# Autodesk Inventor assembly: switchplate-2
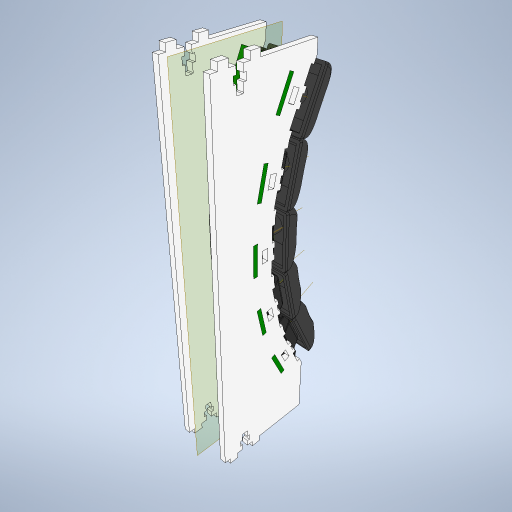
[picture p0: Inventor's stored thumbnail of the model, 512x512]
Saved by Autodesk Inventor 2024.1 (Build 281209000, 209)
## iProperties
Created: 2019-07-06
Part Number: switchplate-2
Document SubType Name: Assembly
Designer: Thibault
Mass: 36.7321 g
Surface Area: 336.688 cm^2
Volume: 13.7102 cm^3
Density: 2.67918 g/cm^3
Author: Thibault
## Documents named in this file (7)
- C:\Users\Thibault\Documents\habilis\mech\switchplate\switchplate-2.iam
- C:\Users\Thibault\Documents\habilis\mech\switchplate_support.ipt
- C:\Users\Thibault Polge\Documents\Habilis\mech\mx.iam
- C:\Users\Thibault\Documents\habilis\mech\mx\DSA-1x1.iam
- C:\Users\Thibault\Documents\habilis\mech\pcb.ipt
- C:\Users\Thibault\Documents\habilis\mech\switchplate.iam
- C:\Users\Thibault\Documents\habilis\mech\switchplate_support\switchplate-support-02.ipt
## Components (12 placed, 4 different names)
1. switchplate-support:left — Affleurement:1, Affleurement:2, Affleurement:3, Affleurement:17, Symétrie:1, Affleurement:23, Placage:1, Placage:3, Placage:6, Placage:7
2. switchplate-support:right — Affleurement:17, Symétrie:1, Affleurement:23, Placage:2, Placage:4, Placage:5, Placage:6, Placage:8, Placage:9, Placage:10, Placage:12, Placage:13, Placage:14, Placage:15, Placage:16, Placage:17, Placage:18, Placage:19, Placage:20, Placage:21, Placage:22, Placage:23, Placage:24, Placage:25, Placage:26, Placage:27, Placage:28, Placage:29, Placage:30, Placage:31, Placage:32
3. Switch:1 [sub-assembly] — Placage:1, Placage:2, Placage:3
4. Switch:2 [sub-assembly] — Placage:8, Placage:9, Placage:10
5. Switch:3 [sub-assembly] — Placage:4, Placage:5, Placage:7
6. Switch:4 [sub-assembly] — Placage:12, Placage:13, Placage:14
7. Switch:5 [sub-assembly] — Placage:15, Placage:16, Placage:17
8. pcb:1 — Placage:21, Placage:31, Placage:32
9. pcb:2 — Placage:22, Placage:29, Placage:30
10. pcb:3 — Placage:19, Placage:27, Placage:28
11. pcb:5 — Placage:20, Placage:23, Placage:24
12. pcb:4 — Placage:18, Placage:25, Placage:26
## Relationships (37: Mate 31, Flush 5, Symmetry 1)
- Affleurement:1 [Flush]: switchplate-support:left
- Affleurement:2 [Flush]: switchplate-support:left
- Affleurement:3 [Flush]: switchplate-support:left
- Affleurement:17 [Flush]: switchplate-support:left ↔ switchplate-support:right
- Symétrie:1 [Symmetry]: switchplate-support:left ↔ switchplate-support:right
- Affleurement:23 [Flush]: switchplate-support:left ↔ switchplate-support:right
- Placage:1 [Mate]: switchplate-support:left ↔ Switch:1
- Placage:2 [Mate]: switchplate-support:right ↔ Switch:1
- Placage:3 [Mate]: switchplate-support:left ↔ Switch:1
- Placage:4 [Mate]: switchplate-support:right ↔ Switch:3
- Placage:5 [Mate]: switchplate-support:right ↔ Switch:3
- Placage:6 [Mate] (14 mm): switchplate-support:left ↔ switchplate-support:right
- Placage:7 [Mate]: switchplate-support:left ↔ Switch:3
- Placage:8 [Mate]: switchplate-support:right ↔ Switch:2
- Placage:9 [Mate]: switchplate-support:right ↔ Switch:2
- Placage:10 [Mate]: switchplate-support:right ↔ Switch:2
- Placage:12 [Mate]: switchplate-support:right ↔ Switch:4
- Placage:13 [Mate]: switchplate-support:right ↔ Switch:4
- Placage:14 [Mate]: switchplate-support:right ↔ Switch:4
- Placage:15 [Mate]: switchplate-support:right ↔ Switch:5
- Placage:16 [Mate]: switchplate-support:right ↔ Switch:5
- Placage:17 [Mate]: switchplate-support:right ↔ Switch:5
- Placage:18 [Mate]: switchplate-support:right ↔ pcb:4
- Placage:19 [Mate]: switchplate-support:right ↔ pcb:3
- Placage:20 [Mate]: switchplate-support:right ↔ pcb:5
- Placage:21 [Mate]: switchplate-support:right ↔ pcb:1
- Placage:22 [Mate]: switchplate-support:right ↔ pcb:2
- Placage:23 [Mate]: switchplate-support:right ↔ pcb:5
- Placage:24 [Mate]: switchplate-support:right ↔ pcb:5
- Placage:25 [Mate]: switchplate-support:right ↔ pcb:4
- Placage:26 [Mate]: switchplate-support:right ↔ pcb:4
- Placage:27 [Mate]: switchplate-support:right ↔ pcb:3
- Placage:28 [Mate]: switchplate-support:right ↔ pcb:3
- Placage:29 [Mate]: switchplate-support:right ↔ pcb:2
- Placage:30 [Mate]: switchplate-support:right ↔ pcb:2
- Placage:31 [Mate]: switchplate-support:right ↔ pcb:1
- Placage:32 [Mate]: switchplate-support:right ↔ pcb:1
